# Autodesk Inventor assembly: UpperBody
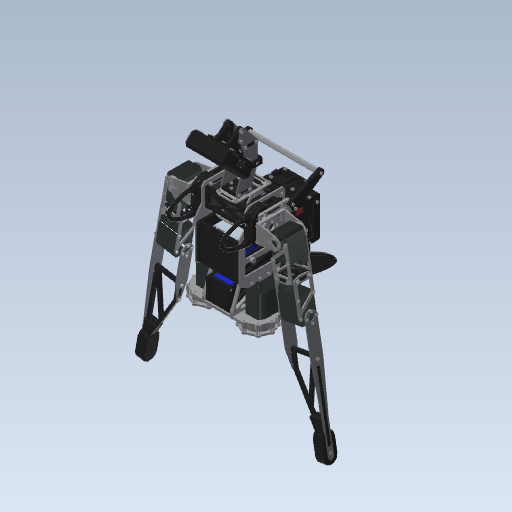
[picture p0: Inventor's stored thumbnail of the model, 512x512]
Saved by Autodesk Inventor 2020.4 (Build 244396000, 396)
## iProperties
Created: 2016-05-03
Part Number: UpperBody
Document SubType Name: Assembly
Designer: hiroaki
Mass: 2450.59 g
Surface Area: 8110.23 cm^2
Volume: 1381.3 cm^3
Density: 1.77412 g/cm^3
Author: hiroaki
## Documents named in this file (7)
- C:\Users\Masato\Documents\Inventor\CIT Brains_Inventor\OpenPlatform_ver3_0 - ver4_0 branch\UpperBody\UpperBody.iam
- C:\Users\Masato\Documents\Inventor\CIT Brains_Inventor\OpenPlatform_ver3_0 - ver4_0 branch\UpperBody\Trunk\Trunk.iam
- C:\Users\Masato\Documents\Inventor\CIT Brains_Inventor\OpenPlatform_ver3_0 - ver4_0 branch\UpperBody\Head\Head.iam
- C:\Users\Masato\Documents\Inventor\CIT Brains_Inventor\OpenPlatform_ver3_0 - ver4_0 branch\UpperBody\Arm\ForeArm.iam
- C:\Users\Masato\Documents\Inventor\CIT Brains_Inventor\OpenPlatform_ver3_0 - ver4_0 branch\UpperBody\Arm\Shoulder.iam
- C:\Users\Masato\Documents\Inventor\CIT Brains_Inventor\OpenPlatform_ver3_0 - ver4_0 branch\UpperBody\Arm\RightUpperArm.iam
- C:\Users\Masato\Documents\Inventor\CIT Brains_Inventor\OpenPlatform_ver3_0 - ver4_0 branch\UpperBody\Arm\LeftUpperArm.iam
## Components (8 placed, 6 different names)
1. Head:1 [sub-assembly] — 挿入:13, 角度:12
2. Trunk:1 [sub-assembly] — 挿入:13, 角度:12, 挿入:22, 挿入:23, フラッシュ:10, 角度:24
3. ForeArm:1 [sub-assembly] — 挿入:87, 角度:25
4. ForeArm:2 [sub-assembly] — 挿入:88, 角度:26
5. RightUpperArm:1 [sub-assembly] — 挿入:88, 挿入:90, 挿入:91, 角度:26
6. LeftUpperArm:1 [sub-assembly] — 挿入:87, 挿入:92, 挿入:93, 角度:25
7. Shoulder:1 [sub-assembly] — 挿入:22, 角度:23, 角度:24, 挿入:92, 挿入:93
8. Shoulder:2 [sub-assembly] — 挿入:23, 角度:23, 挿入:90, 挿入:91
## Relationships (15: Insert 9, Angle 5, Flush 1)
- 挿入:13 [Insert]: Head:1 ↔ Trunk:1
- 角度:12 [Angle] (0 deg): Head:1 ↔ Trunk:1
- 挿入:22 [Insert]: Trunk:1 ↔ Shoulder:1
- 挿入:23 [Insert]: Trunk:1 ↔ Shoulder:2
- 角度:23 [Angle] (0 deg): Shoulder:1 ↔ Shoulder:2
- フラッシュ:10 [Flush]: Trunk:1
- 挿入:87 [Insert]: ForeArm:1 ↔ LeftUpperArm:1
- 挿入:88 [Insert]: ForeArm:2 ↔ RightUpperArm:1
- 角度:24 [Angle] (0 deg): Trunk:1 ↔ Shoulder:1
- 挿入:90 [Insert]: RightUpperArm:1 ↔ Shoulder:2
- 挿入:91 [Insert]: RightUpperArm:1 ↔ Shoulder:2
- 挿入:92 [Insert]: LeftUpperArm:1 ↔ Shoulder:1
- 挿入:93 [Insert]: LeftUpperArm:1 ↔ Shoulder:1
- 角度:25 [Angle] (0 deg): ForeArm:1 ↔ LeftUpperArm:1
- 角度:26 [Angle] (0 deg): ForeArm:2 ↔ RightUpperArm:1
